# Autodesk Inventor assembly: Singel doodr
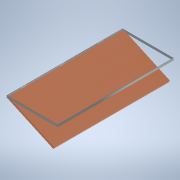
[picture p0: Inventor's stored thumbnail of the model, 180x180]
Saved by Autodesk Inventor 2021 (Build 250183000, 183)
## iProperties
Created: 2021-07-31
Part Number: Singel doodr
Document SubType Name: Assembly
Designer: Shammy Haider
Author: Shammy Haider
## Documents named in this file (4)
- D:\Designing\Autodesk inventor\Wood Door\Singel doodr.iam
- D:\Designing\Autodesk inventor\Wood Door\Frame1.ipt
- D:\Designing\Autodesk inventor\Wood Door\Door.ipt
- D:\Designing\Autodesk inventor\Wood Door\Hinge assembly.iam
## Components (5 placed, 3 different names)
1. Frame1:1 — Mate:1, Mate:2, Mate:3, Mate:4, Mate:5, Mate:6, Mate:7, Angle:1
2. Door:1 — Mate:11, Mate:12, Mate:13, Mate:14, Mate:15, Mate:16, Mate:17
3. Hinge assembly:1 [sub-assembly] — Mate:1, Mate:2, Mate:8, Mate:13, Mate:16
4. Hinge assembly:2 [sub-assembly] — Mate:3, Mate:6, Mate:9, Mate:12, Mate:15, Mate:17
5. Hinge assembly:3 [sub-assembly] — Mate:4, Mate:5, Mate:10, Mate:11, Mate:14
## Relationships (18: Mate 17, Angle 1)
- Mate:1: Frame1:1 ↔ Hinge assembly:1
- Mate:2: Frame1:1 ↔ Hinge assembly:1
- Mate:3: Frame1:1 ↔ Hinge assembly:2
- Mate:4: Frame1:1 ↔ Hinge assembly:3
- Mate:5: Frame1:1 ↔ Hinge assembly:3
- Mate:6: Frame1:1 ↔ Hinge assembly:2
- Mate:7: Frame1:1
- Angle:1 (180 deg): Frame1:1
- Mate:8: Hinge assembly:1
- Mate:9: Hinge assembly:2
- Mate:10: Hinge assembly:3
- Mate:11: Door:1 ↔ Hinge assembly:3
- Mate:12: Door:1 ↔ Hinge assembly:2
- Mate:13: Door:1 ↔ Hinge assembly:1
- Mate:14: Door:1 ↔ Hinge assembly:3
- Mate:15: Door:1 ↔ Hinge assembly:2
- Mate:16: Door:1 ↔ Hinge assembly:1
- Mate:17: Door:1 ↔ Hinge assembly:2
